# Autodesk Inventor assembly: Final Assembly
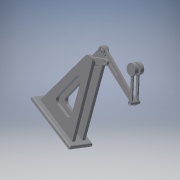
[picture p0: Inventor's stored thumbnail of the model, 180x180]
Saved by Autodesk Inventor 2017.1 (Build 211199000, 199)
## iProperties
Created: 2017-05-25
Part Number: Final Assembly
Document SubType Name: Assembly
Designer: 196918
Author: 196918
## Documents named in this file (9)
- C:\Users\196918.FCBOE\Desktop\2017 engi final exam Bibby\Final Assembly.iam
- C:\Users\196918.FCBOE\Desktop\2017 engi final exam Bibby\Crank.ipt
- C:\Users\196918.FCBOE\Desktop\2017 engi final exam Bibby\lever.ipt
- C:\Users\196918.FCBOE\Desktop\2017 engi final exam Bibby\pendulum.ipt
- C:\Users\196918.FCBOE\Desktop\2017 engi final exam Bibby\shaft 6x24.ipt
- C:\Users\196918.FCBOE\Desktop\2017 engi final exam Bibby\shaft 6x24-1.ipt
- C:\Users\196918.FCBOE\Desktop\2017 engi final exam Bibby\shaft 6x24-2.ipt
- C:\Users\196918.FCBOE\Desktop\2017 engi final exam Bibby\Stand.ipt
- C:\Users\196918.FCBOE\Desktop\2017 engi final exam Bibby\pendulum_MIR.ipt
## Components (9 placed, 8 different names)
1. Crank:1 — Rotational:2, Rotational:3
2. lever:1 — Rotational:4, Cylindrical:1
3. pendulum:1 — Rotational:5
4. shaft 6x24:1 — Rigid:1, Rotational:4
5. shaft 6x24-1:1 — Rotational:1, Rotational:2
6. shaft 6x24-2:1 — Rotational:3
7. Stand:1 — Rotational:1, Rigid:1
8. shaft 6x24-1:2 — Cylindrical:1, Rotational:5
9. pendulum_MIR:1
## Relationships (7: RevoluteJoint 5, WeldJoint 1, CylindricalJoint 1)
- Rotational:1 [RevoluteJoint]: shaft 6x24-1:1 ↔ Stand:1
- Rotational:2 [RevoluteJoint]: Crank:1 ↔ shaft 6x24-1:1
- Rotational:3 [RevoluteJoint]: Crank:1 ↔ shaft 6x24-2:1
- Rigid:1 [WeldJoint]: shaft 6x24:1 ↔ Stand:1
- Rotational:4 [RevoluteJoint]: lever:1 ↔ shaft 6x24:1
- Cylindrical:1: lever:1 ↔ shaft 6x24-1:2
- Rotational:5 [RevoluteJoint]: pendulum:1 ↔ shaft 6x24-1:2
